# Autodesk Inventor assembly: Kiwi Robot
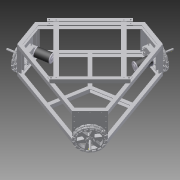
[picture p0: Inventor's stored thumbnail of the model, 180x180]
Saved by Autodesk Inventor 2013 (Build 170138000, 138)
## iProperties
Created: 2013-01-29
Part Number: Kiwi Robot
Document SubType Name: Assembly
Designer: carneeki
Author: carneeki
## Documents named in this file (5)
- C:\Users\carneeki\Desktop\Kiwi Robot\Kiwi Robot.iam
- C:\Users\carneeki\Desktop\Kiwi Robot\Chassis\Chassis.iam
- C:\Users\carneeki\Desktop\Kiwi Robot\Ground.ipt
- C:\Users\carneeki\Desktop\Kiwi Robot\Drive Wheel\Drive Wheel.iam
- C:\Users\carneeki\Desktop\Kiwi Robot\Rack\Rack.iam
## Components (6 placed, 4 different names)
1. Chassis:1 [sub-assembly] — Mate:1, Mate:2, Flush:1, Flush:2, Mate:3, Flush:3, Flush:4, Mate:4, Flush:5, Flush:6, Flush:9, Insert:1, Insert:2
2. Ground:1 — Mate:1, Flush:9
3. Rack:1 [sub-assembly] — Insert:1, Insert:2
4. Drive Wheel:1 [sub-assembly] — Mate:2, Flush:1, Flush:2
5. Drive Wheel:2 [sub-assembly] — Mate:4, Flush:5, Flush:6
6. Drive Wheel:3 [sub-assembly] — Mate:3, Flush:3, Flush:4
## Relationships (13: Flush 7, Mate 4, Insert 2)
- Mate:1 (38.1 mm): Chassis:1 ↔ Ground:1
- Mate:2: Chassis:1 ↔ Drive Wheel:1
- Flush:1: Chassis:1 ↔ Drive Wheel:1
- Flush:2: Chassis:1 ↔ Drive Wheel:1
- Mate:3: Chassis:1 ↔ Drive Wheel:3
- Flush:3: Chassis:1 ↔ Drive Wheel:3
- Flush:4: Chassis:1 ↔ Drive Wheel:3
- Mate:4: Chassis:1 ↔ Drive Wheel:2
- Flush:5: Chassis:1 ↔ Drive Wheel:2
- Flush:6: Chassis:1 ↔ Drive Wheel:2
- Flush:9 (254 mm): Chassis:1 ↔ Ground:1
- Insert:1: Chassis:1 ↔ Rack:1
- Insert:2: Chassis:1 ↔ Rack:1
